# Autodesk Inventor assembly: Flanged Ball Valve - 50NB PN16
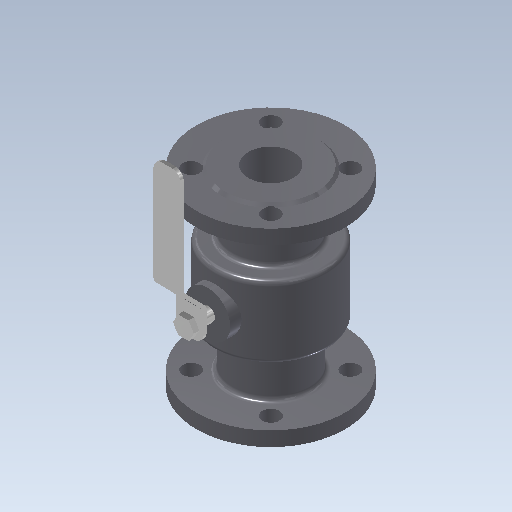
[picture p0: Inventor's stored thumbnail of the model, 512x512]
Saved by Autodesk Inventor 2020 (Build 240168000, 168)
## iProperties
Created: 2009-08-10
Part Number: Flanged Ball Valve - 50NB PN16
Document SubType Name: Assembly
Designer: Demir Ali
Description: Flanged Ball Valve - 50NB PN16
Stock Number: NA
Author: Demir Ali
Title: Purchased Part
Revision Number: A
## Documents named in this file (3)
- C:\Users\akensoa\OneDrive - autodesk\Models\Process Equipment\Workspace\Supplier Content\Valves\Flanged Ball Valve - 50NB PN16.iam
- C:\Users\akensoa\OneDrive - autodesk\Models\Process Equipment\Workspace\Supplier Content\Valves\Flanged Ball Valve - 50NB PN16.ipt
- C:\Users\akensoa\OneDrive - autodesk\Models\Process Equipment\Workspace\Supplier Content\Valves\Flanged Ball Valve Handle - 50NB PN16.ipt
## Components (2 placed, 2 different names)
1. Flanged Ball Valve - 50NB PN16:1 — Insert:1
2. Flanged Ball Valve Handle - 50NB PN16:1 — Insert:1
## Relationships (1: Insert 1)
- Insert:1: Flanged Ball Valve - 50NB PN16:1 ↔ Flanged Ball Valve Handle - 50NB PN16:1
